# Autodesk Inventor assembly: arm stop + switch
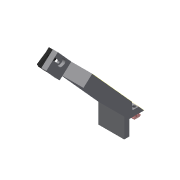
[picture p0: Inventor's stored thumbnail of the model, 180x180]
Saved by Autodesk Inventor 2018 (Build 220112000, 112)
## iProperties
Created: 2018-12-28
Part Number: arm stop + switch
Document SubType Name: Assembly
Designer: ball
Author: ball
## Documents named in this file (5)
- C:\FTC\FTC8863CAD\2018Robot\arm stop + switch.iam
- C:\FTC\FTC8863CAD\Actobotics\585 parts\585718.ipt
- C:\FTC\FTC8863CAD\Actobotics\565 parts\565150.ipt
- C:\FTC\FTC8863CAD\2018Robot\arm stop.ipt
- C:\FTC\FTC8863CAD\Actobotics\605 parts\605630.ipt
## Components (4 placed, 4 different names)
1. 565150:1 — Mate:1, Mate:2, Flush:1
2. 585718:2 — Mate:1, Mate:2, Flush:1, Flush:2
3. arm stop:1 — Flush:2, Mate:3, Flush:3, Flush:4
4. 605630:1 — Mate:3, Flush:3, Flush:4
## Relationships (7: Flush 4, Mate 3)
- Mate:1: 565150:1 ↔ 585718:2
- Mate:2: 565150:1 ↔ 585718:2
- Flush:1 (25.4 mm): 565150:1 ↔ 585718:2
- Flush:2: 585718:2 ↔ arm stop:1
- Mate:3: arm stop:1 ↔ 605630:1
- Flush:3 (2.54 mm): arm stop:1 ↔ 605630:1
- Flush:4: arm stop:1 ↔ 605630:1
